# Autodesk Inventor assembly: КВ33.044.500 - Каретка оси Y
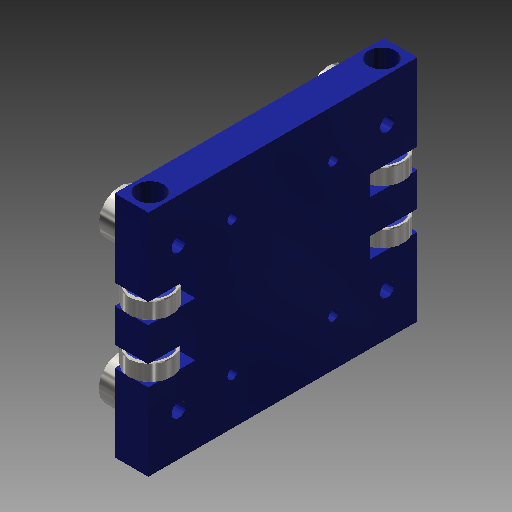
[picture p0: Inventor's stored thumbnail of the model, 512x512]
Saved by Autodesk Inventor 2019 (Build 230136000, 136)
## iProperties
Created: 2019-07-21
Part Number: КВ33.044.500 - Каретка оси Y
Material: Типовые
Document SubType Name: Assembly
Designer: Петров Иван
Author: Петров Иван
## Documents named in this file (3)
- C:\Users\user\Documents\Kvantoriada2019\optimal_gripper\hardware\КВ33.044.600 - Каретка оси Y.iam
- C:\Users\user\Documents\Kvantoriada2019\optimal_gripper\hardware\КВ33.044.601 - Щека каретка оси Y.ipt
- C:\Users\user\Documents\Kvantoriada2019\optimal_gripper\hardware\Стандартные изделия\Подшипник 624Z.ipt
## Components (9 placed, 2 different names)
1. КВ33.044.601 - Щека каретка оси Y:1 — Совмещение:1, Совмещение:2, Совмещение:3, Совмещение:4, Совмещение:5, Совмещение:6, 2.5, Совмещение:8, Совмещение:9, Совмещение:10, Совмещение:11, Совмещение:12, Совмещение:13, Совмещение:14, Совмещение:15, Совмещение:16
2. Подшипник 624Z:1 — Совмещение:1, Совмещение:8
3. Подшипник 624Z:2 — Совмещение:4, Совмещение:5
4. Подшипник 624Z:3 — Совмещение:3, Совмещение:6
5. Подшипник 624Z:4 — Совмещение:2, 2.5
6. Подшипник 624Z:5 — Совмещение:9, Совмещение:15
7. Подшипник 624Z:6 — Совмещение:10, Совмещение:16
8. Подшипник 624Z:7 — Совмещение:11, Совмещение:13
9. Подшипник 624Z:8 — Совмещение:12, Совмещение:14
## Relationships (16: Mate 16)
- Совмещение:1 [Mate]: КВ33.044.601 - Щека каретка оси Y:1 ↔ Подшипник 624Z:1
- Совмещение:2 [Mate]: КВ33.044.601 - Щека каретка оси Y:1 ↔ Подшипник 624Z:4
- Совмещение:3 [Mate]: КВ33.044.601 - Щека каретка оси Y:1 ↔ Подшипник 624Z:3
- Совмещение:4 [Mate]: КВ33.044.601 - Щека каретка оси Y:1 ↔ Подшипник 624Z:2
- Совмещение:5 [Mate] (2.5 mm): КВ33.044.601 - Щека каретка оси Y:1 ↔ Подшипник 624Z:2
- Совмещение:6 [Mate] (2.5 mm): КВ33.044.601 - Щека каретка оси Y:1 ↔ Подшипник 624Z:3
- 2.5 [Mate] (2.5 mm): КВ33.044.601 - Щека каретка оси Y:1 ↔ Подшипник 624Z:4
- Совмещение:8 [Mate] (2.5 mm): КВ33.044.601 - Щека каретка оси Y:1 ↔ Подшипник 624Z:1
- Совмещение:9 [Mate]: КВ33.044.601 - Щека каретка оси Y:1 ↔ Подшипник 624Z:5
- Совмещение:10 [Mate]: КВ33.044.601 - Щека каретка оси Y:1 ↔ Подшипник 624Z:6
- Совмещение:11 [Mate]: КВ33.044.601 - Щека каретка оси Y:1 ↔ Подшипник 624Z:7
- Совмещение:12 [Mate]: КВ33.044.601 - Щека каретка оси Y:1 ↔ Подшипник 624Z:8
- Совмещение:13 [Mate] (0.5 mm): КВ33.044.601 - Щека каретка оси Y:1 ↔ Подшипник 624Z:7
- Совмещение:14 [Mate] (0.5 mm): КВ33.044.601 - Щека каретка оси Y:1 ↔ Подшипник 624Z:8
- Совмещение:15 [Mate] (0.5 mm): КВ33.044.601 - Щека каретка оси Y:1 ↔ Подшипник 624Z:5
- Совмещение:16 [Mate] (0.5 mm): КВ33.044.601 - Щека каретка оси Y:1 ↔ Подшипник 624Z:6
